# Autodesk Inventor assembly: Cartridge Tube Seal
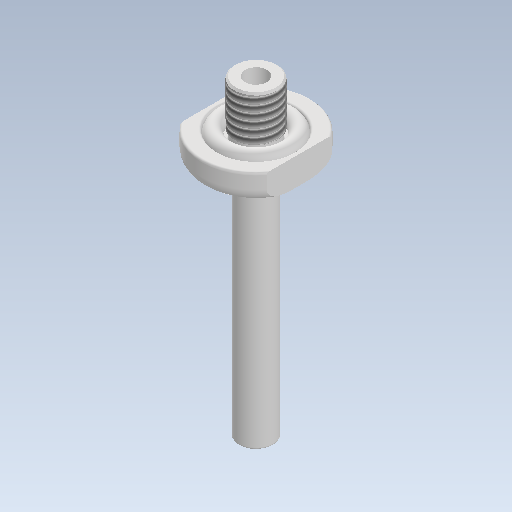
[picture p0: Inventor's stored thumbnail of the model, 512x512]
Saved by Autodesk Inventor 2021 (Build 250183000, 183)
## iProperties
Created: 2020-04-22
Part Number: Cartridge Tube Seal
Document SubType Name: Assembly
Designer: jgray
Author: jgray
## Documents named in this file (3)
- M:\Printed Electronics\Gas Sensors\Prototypes\Prototype II - Cartridge Reader\Full Cart Interface V3 28-5-20\Workspaces\Workspace\Workspaces\Workspace\Cartridge Tube Seal.iam
- M:\Printed Electronics\Gas Sensors\Prototypes\Prototype II - Cartridge Reader\Full Cart Interface V3 28-5-20\Workspaces\Workspace\Workspaces\Workspace\Cartridge Interface Tube.ipt
- M:\Printed Electronics\Gas Sensors\Prototypes\Prototype II - Cartridge Reader\Full Cart Interface V3 28-5-20\Workspaces\Workspace\Workspaces\Workspace\RS 527-9778 Si-O-Ring 5-28ID 1-79 THK 11-32INCH OD.ipt
## Components (2 placed, 2 different names)
1. Cartridge Interface Tube:1 — Mate:1, Tangent:1
2. RS 527-9778 Si-O-Ring 5-28ID 1-79 THK 11-32INCH OD:1 — Mate:1, Tangent:1
## Relationships (2: Mate 1, Tangent 1)
- Mate:1: Cartridge Interface Tube:1 ↔ RS 527-9778 Si-O-Ring 5-28ID 1-79 THK 11-32INCH OD:1
- Tangent:1: Cartridge Interface Tube:1 ↔ RS 527-9778 Si-O-Ring 5-28ID 1-79 THK 11-32INCH OD:1
